# Autodesk Inventor assembly: Bottom PVC Roller
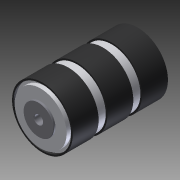
[picture p0: Inventor's stored thumbnail of the model, 180x180]
Saved by Autodesk Inventor 2014 SP1 (Build 180222100, 222)
## iProperties
Created: 2012-03-30
Part Number: Bottom PVC Roller
Document SubType Name: Assembly
Designer: Moses
Author: Moses
## Documents named in this file (5)
- C:\Users\Moses\Documents\Inventor\Rebuild\Repackaged_Team 3061_2012 Ball Shooter_Inventor Version_2014\Bottom PVC Roller.iam
- C:\Users\Moses\Documents\Inventor\Rebuild\Repackaged_Team 3061_2012 Ball Shooter_Inventor Version_2014\PVC Cap.ipt
- C:\Users\Moses\Documents\Inventor\Rebuild\Repackaged_Team 3061_2012 Ball Shooter_Inventor Version_2014\0.25 in Flanged Ball Bearing.ipt
- C:\Users\Moses\Documents\Inventor\Rebuild\Repackaged_Team 3061_2012 Ball Shooter_Inventor Version_2014\V5 Shooter Conveyor Roller.ipt
- C:\Users\Moses\Documents\Inventor\Rebuild\Repackaged_Team 3061_2012 Ball Shooter_Inventor Version_2014\PVC Rubber Covering.ipt
## Components (8 placed, 4 different names)
1. PVC Cap:1 — Insert:1, Insert:3
2. PVC Cap:2 — Insert:2, Insert:4
3. 0.25 in Flanged Ball Bearing:1 — Insert:1
4. 0.25 in Flanged Ball Bearing:2 — Insert:2
5. V5 Shooter Conveyor Roller:1 — Insert:3, Insert:4, Mate:1, Mate:2, Mate:3, Flush:1
6. PVC Rubber Covering:1 — Mate:2, Mate:4, Mate:5, Flush:1
7. PVC Rubber Covering:2 — Mate:1, Mate:4
8. PVC Rubber Covering:3 — Mate:3, Mate:5
## Relationships (10: Mate 5, Insert 4, Flush 1)
- Insert:1: PVC Cap:1 ↔ 0.25 in Flanged Ball Bearing:1
- Insert:2: PVC Cap:2 ↔ 0.25 in Flanged Ball Bearing:2
- Insert:3: PVC Cap:1 ↔ V5 Shooter Conveyor Roller:1
- Insert:4: PVC Cap:2 ↔ V5 Shooter Conveyor Roller:1
- Mate:1: V5 Shooter Conveyor Roller:1 ↔ PVC Rubber Covering:2
- Mate:2: V5 Shooter Conveyor Roller:1 ↔ PVC Rubber Covering:1
- Mate:3: V5 Shooter Conveyor Roller:1 ↔ PVC Rubber Covering:3
- Mate:4 (6.35 mm): PVC Rubber Covering:1 ↔ PVC Rubber Covering:2
- Mate:5 (6.35 mm): PVC Rubber Covering:1 ↔ PVC Rubber Covering:3
- Flush:1 (23.495 mm): V5 Shooter Conveyor Roller:1 ↔ PVC Rubber Covering:1
